# Autodesk Inventor assembly: Skateboard Box
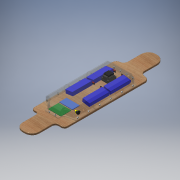
[picture p0: Inventor's stored thumbnail of the model, 180x180]
Saved by Autodesk Inventor 2017.3 (Build 213256000, 256)
## iProperties
Created: 2019-01-10
Part Number: Skateboard Box
Document SubType Name: Assembly
Designer: LSabe
Author: LSabe
## Documents named in this file (11)
- C:\Users\LSabe\OneDrive\Documents\Skateboard Box Files\Skateboard Box.iam
- C:\Users\LSabe\OneDrive\Documents\Skateboard Box Files\ESC.ipt
- C:\Users\LSabe\OneDrive\Documents\Inventor\Content Center Files\R2017\en-US\ANSI B18.6.3(03)\ANSI B18.6.3 - 10-32 UNF - 0.75(14).ipt
- C:\Users\LSabe\OneDrive\Documents\Skateboard Box Files\Battery.ipt
- C:\Users\LSabe\OneDrive\Documents\Skateboard Box Files\Lipo Charger Circuit.ipt
- C:\Users\LSabe\OneDrive\Documents\Skateboard Box Files\Receiver PCB.ipt
- C:\Users\LSabe\OneDrive\Documents\Skateboard Box Files\Power Switch.ipt
- C:\Users\LSabe\OneDrive\Documents\Skateboard Box Files\Skateboard Deck.ipt
- C:\Users\LSabe\OneDrive\Documents\Skateboard Box Files\Skateboard Box Back.ipt
- C:\Users\LSabe\OneDrive\Documents\Skateboard Box Files\Skateboard Box Front.ipt
- C:\Users\LSabe\OneDrive\Documents\Skateboard Box Files\Skateboard Box Middle.ipt
## Components (30 placed, 10 different names)
1. ESC:1 — Mate:16, Mate:20, Flush:10
2. Receiver PCB:1 — Mate:15, Mate:17, Mate:43
3. Battery:1 — Mate:13, Flush:2, Flush:3
4. Battery:2 — Mate:14, Flush:2, Flush:4
5. Battery:3 — Mate:11, Flush:1, Flush:4
6. Battery:4 — Mate:12, Flush:1, Flush:3
7. Power Switch:1 — Mate:44, Flush:8, Flush:9
8. Skateboard Deck:1 — Mate:11, Mate:12, Mate:13, Mate:14, Mate:15, Mate:16, Mate:17, Mate:20, Mate:21, Mate:22, Mate:23, Mate:24, Flush:5, Mate:45
9. Lipo Charger Circuit:1 — Mate:21, Mate:45
10. Skateboard Box Front:1 — Mate:24, Flush:7, Mate:25, Mate:27, Mate:28, Mate:29, Mate:35, Mate:38, Mate:40, Mate:43, Mate:44, Flush:8, Flush:9
11. Skateboard Box Middle:1 — Mate:23, Flush:5, Flush:6, Flush:7, Mate:25, Mate:26, Mate:31, Mate:33, Mate:36, Mate:41
12. Skateboard Box Back:1 — Mate:22, Flush:6, Mate:26, Mate:30, Mate:32, Mate:34, Mate:37, Mate:39, Mate:42, Flush:10
13. Cross Recessed Binding Head Machine Screw - Type I - Inch No. 10 - 32 - 3/4:22 — Mate:28, Mate:35
14. Cross Recessed Binding Head Machine Screw - Type I - Inch No. 10 - 32 - 3/4:27
15. Cross Recessed Binding Head Machine Screw - Type I - Inch No. 10 - 32 - 3/4:24 — Mate:31, Mate:36
16. Cross Recessed Binding Head Machine Screw - Type I - Inch No. 10 - 32 - 3/4:28
17. Cross Recessed Binding Head Machine Screw - Type I - Inch No. 10 - 32 - 3/4:25 — Mate:32, Mate:37
18. Cross Recessed Binding Head Machine Screw - Type I - Inch No. 10 - 32 - 3/4:29
19. Cross Recessed Binding Head Machine Screw - Type I - Inch No. 10 - 32 - 3/4:20 — Mate:29, Mate:40
20. Cross Recessed Binding Head Machine Screw - Type I - Inch No. 10 - 32 - 3/4:30
21. Cross Recessed Binding Head Machine Screw - Type I - Inch No. 10 - 32 - 3/4:26 — Mate:33, Mate:41
22. Cross Recessed Binding Head Machine Screw - Type I - Inch No. 10 - 32 - 3/4:31
23. Cross Recessed Binding Head Machine Screw - Type I - Inch No. 10 - 32 - 3/4:23 — Mate:34, Mate:42
24. Cross Recessed Binding Head Machine Screw - Type I - Inch No. 10 - 32 - 3/4:32
25. Cross Recessed Binding Head Machine Screw - Type I - Inch No. 10 - 32 - 3/4:21 — Mate:30, Mate:39
26. Cross Recessed Binding Head Machine Screw - Type I - Inch No. 10 - 32 - 3/4:33
27. Cross Recessed Binding Head Machine Screw - Type I - Inch No. 10 - 32 - 3/4:34
28. Cross Recessed Binding Head Machine Screw - Type I - Inch No. 10 - 32 - 3/4:35
29. Cross Recessed Binding Head Machine Screw - Type I - Inch No. 10 - 32 - 3/4:19 — Mate:27, Mate:38
30. Cross Recessed Binding Head Machine Screw - Type I - Inch No. 10 - 32 - 3/4:36
## Component patterns: (2 elements, first: Cross Recessed Binding Head Machine Screw - Type I - Inch No. 10 - 32 - 3/4:22), (2 elements, first: Cross Recessed Binding Head Machine Screw - Type I - Inch No. 10 - 32 - 3/4:24), (2 elements, first: Cross Recessed Binding Head Machine Screw - Type I - Inch No. 10 - 32 - 3/4:25), (2 elements, first: Cross Recessed Binding Head Machine Screw - Type I - Inch No. 10 - 32 - 3/4:20), (2 elements, first: Cross Recessed Binding Head Machine Screw - Type I - Inch No. 10 - 32 - 3/4:26), (2 elements, first: Cross Recessed Binding Head Machine Screw - Type I - Inch No. 10 - 32 - 3/4:23), (4 elements, first: Cross Recessed Binding Head Machine Screw - Type I - Inch No. 10 - 32 - 3/4:21), (2 elements, first: Cross Recessed Binding Head Machine Screw - Type I - Inch No. 10 - 32 - 3/4:19)
## Relationships (43: Mate 33, Flush 10)
- Mate:11: Battery:3 ↔ Skateboard Deck:1
- Mate:12: Battery:4 ↔ Skateboard Deck:1
- Mate:13: Battery:1 ↔ Skateboard Deck:1
- Mate:14: Battery:2 ↔ Skateboard Deck:1
- Mate:15: Receiver PCB:1 ↔ Skateboard Deck:1
- Mate:16 (8.89 mm): ESC:1 ↔ Skateboard Deck:1
- Flush:1: Battery:3 ↔ Battery:4
- Flush:2: Battery:1 ↔ Battery:2
- Flush:3: Battery:1 ↔ Battery:4
- Flush:4: Battery:2 ↔ Battery:3
- Mate:17: Receiver PCB:1 ↔ Skateboard Deck:1
- Mate:20: ESC:1 ↔ Skateboard Deck:1
- Mate:21: Skateboard Deck:1 ↔ Lipo Charger Circuit:1
- Mate:22: Skateboard Deck:1 ↔ Skateboard Box Back:1
- Mate:23: Skateboard Deck:1 ↔ Skateboard Box Middle:1
- Mate:24: Skateboard Deck:1 ↔ Skateboard Box Front:1
- Flush:5: Skateboard Deck:1 ↔ Skateboard Box Middle:1
- Flush:6: Skateboard Box Middle:1 ↔ Skateboard Box Back:1
- Flush:7: Skateboard Box Front:1 ↔ Skateboard Box Middle:1
- Mate:25: Skateboard Box Front:1 ↔ Skateboard Box Middle:1
- Mate:26: Skateboard Box Middle:1 ↔ Skateboard Box Back:1
- Mate:27: Skateboard Box Front:1 ↔ Cross Recessed Binding Head Machine Screw - Type I - Inch No. 10 - 32 - 3/4:19
- Mate:28: Skateboard Box Front:1 ↔ Cross Recessed Binding Head Machine Screw - Type I - Inch No. 10 - 32 - 3/4:22
- Mate:29: Skateboard Box Front:1 ↔ Cross Recessed Binding Head Machine Screw - Type I - Inch No. 10 - 32 - 3/4:20
- Mate:30: Skateboard Box Back:1 ↔ Cross Recessed Binding Head Machine Screw - Type I - Inch No. 10 - 32 - 3/4:21
- Mate:31: Skateboard Box Middle:1 ↔ Cross Recessed Binding Head Machine Screw - Type I - Inch No. 10 - 32 - 3/4:24
- Mate:32: Skateboard Box Back:1 ↔ Cross Recessed Binding Head Machine Screw - Type I - Inch No. 10 - 32 - 3/4:25
- Mate:33: Skateboard Box Middle:1 ↔ Cross Recessed Binding Head Machine Screw - Type I - Inch No. 10 - 32 - 3/4:26
- Mate:34: Skateboard Box Back:1 ↔ Cross Recessed Binding Head Machine Screw - Type I - Inch No. 10 - 32 - 3/4:23
- Mate:35: Skateboard Box Front:1 ↔ Cross Recessed Binding Head Machine Screw - Type I - Inch No. 10 - 32 - 3/4:22
- Mate:36: Skateboard Box Middle:1 ↔ Cross Recessed Binding Head Machine Screw - Type I - Inch No. 10 - 32 - 3/4:24
- Mate:37: Skateboard Box Back:1 ↔ Cross Recessed Binding Head Machine Screw - Type I - Inch No. 10 - 32 - 3/4:25
- Mate:38: Skateboard Box Front:1 ↔ Cross Recessed Binding Head Machine Screw - Type I - Inch No. 10 - 32 - 3/4:19
- Mate:39: Skateboard Box Back:1 ↔ Cross Recessed Binding Head Machine Screw - Type I - Inch No. 10 - 32 - 3/4:21
- Mate:40: Skateboard Box Front:1 ↔ Cross Recessed Binding Head Machine Screw - Type I - Inch No. 10 - 32 - 3/4:20
- Mate:41: Skateboard Box Middle:1 ↔ Cross Recessed Binding Head Machine Screw - Type I - Inch No. 10 - 32 - 3/4:26
- Mate:42: Skateboard Box Back:1 ↔ Cross Recessed Binding Head Machine Screw - Type I - Inch No. 10 - 32 - 3/4:23
- Mate:43 (3.81 mm): Receiver PCB:1 ↔ Skateboard Box Front:1
- Mate:44: Power Switch:1 ↔ Skateboard Box Front:1
- Flush:8 (25.0952 mm): Power Switch:1 ↔ Skateboard Box Front:1
- Flush:9 (-66.675 mm): Power Switch:1 ↔ Skateboard Box Front:1
- Flush:10 (63.5 mm): ESC:1 ↔ Skateboard Box Back:1
- Mate:45: Skateboard Deck:1 ↔ Lipo Charger Circuit:1
